# Autodesk Inventor assembly: servo_link_assembly
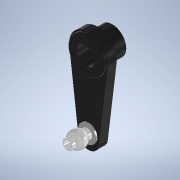
[picture p0: Inventor's stored thumbnail of the model, 180x180]
Saved by Autodesk Inventor 2020 (Build 240168000, 168)
## iProperties
Created: 2019-12-03
Part Number: servo_link_assembly
Document SubType Name: Assembly
Designer: maste
Author: maste
## Documents named in this file (4)
- C:\Users\maste\Documents\GitHub\autobot\robot_model\servo_link_assembly.iam
- C:\Users\maste\Documents\GitHub\autobot\robot_model\RCT-P070_servo_linkage.ipt
- C:\Users\maste\Documents\GitHub\autobot\robot_model\RCT-H022_washer_31_60_05.ipt
- C:\Users\maste\Documents\GitHub\autobot\robot_model\H016.ipt
## Components (3 placed, 3 different names)
1. RCT-P070_servo_linkage:1 — Mate:1, Mate:2, Mate:3
2. RCT-H022_washer_31_60_05:1 — Mate:1, Mate:2, Mate:4
3. H016:1 — Mate:3, Mate:4
## Relationships (4: Mate 4)
- Mate:1: RCT-P070_servo_linkage:1 ↔ RCT-H022_washer_31_60_05:1
- Mate:2: RCT-P070_servo_linkage:1 ↔ RCT-H022_washer_31_60_05:1
- Mate:3: RCT-P070_servo_linkage:1 ↔ H016:1
- Mate:4: RCT-H022_washer_31_60_05:1 ↔ H016:1
